# Autodesk Inventor assembly: Z-head-assembly-HiWin-MGN07
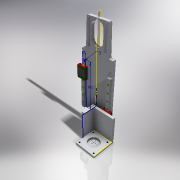
[picture p0: Inventor's stored thumbnail of the model, 180x180]
Saved by Autodesk Inventor 2016 (Build 200138000, 138)
## iProperties
Created: 2015-04-22
Part Number: Z-head-assembly-HiWin-MGN07
Document SubType Name: Assembly
Designer: ax
Author: ax
## Documents named in this file (4)
- C:\Users\ax\Documents\Inventor\mintplacer\Z-head-assembly.iam
- C:\Users\ax\Documents\Inventor\mintplacer\Z-baseplate.ipt
- C:\Users\ax\Documents\Inventor\mintplacer\MGN07C_1_R_80_ZF_H_M_1.iam
- C:\Users\ax\Documents\Inventor\mintplacer\head-assembly.iam
## Components (4 placed, 3 different names)
1. Z-baseplate:1 — Mate:1, Mate:2, Mate:3, Flush:1, Mate:4, Flush:3
2. MGN07C_1_R_80_ZF_H_M_1:1 [sub-assembly] — Mate:1, Mate:2, Mate:3
3. MGN07C_1_R_80_ZF_H_M_1:2 [sub-assembly] — Flush:1, Mate:4, Flush:2
4. head-assembly:1 [sub-assembly] — Flush:2, Flush:3
## Relationships (7: Mate 4, Flush 3)
- Mate:1: Z-baseplate:1 ↔ MGN07C_1_R_80_ZF_H_M_1:1
- Mate:2: Z-baseplate:1 ↔ MGN07C_1_R_80_ZF_H_M_1:1
- Mate:3: Z-baseplate:1 ↔ MGN07C_1_R_80_ZF_H_M_1:1
- Flush:1: Z-baseplate:1 ↔ MGN07C_1_R_80_ZF_H_M_1:2
- Mate:4: Z-baseplate:1 ↔ MGN07C_1_R_80_ZF_H_M_1:2
- Flush:2: MGN07C_1_R_80_ZF_H_M_1:2 ↔ head-assembly:1
- Flush:3 (4 mm): Z-baseplate:1 ↔ head-assembly:1
